# Autodesk Inventor assembly: Assembly3
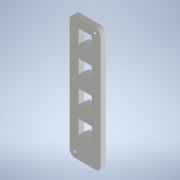
[picture p0: Inventor's stored thumbnail of the model, 180x180]
Saved by Autodesk Inventor 2020 (Build 240168000, 168)
## iProperties
Created: 2019-05-06
Part Number: Assembly3
Document SubType Name: Assembly
Designer: erwin
Author: erwin
## Documents named in this file (3)
- D:\GitHub\ProtoSwitchBoard\design\pin-header_cutter\Assembly3.iam
- D:\GitHub\ProtoSwitchBoard\design\pin-header_cutter\open_side.ipt
- D:\GitHub\ProtoSwitchBoard\design\pin-header_cutter\close_side.ipt
## Components (2 placed, 2 different names)
1. open_side:1 — Rigid:1
2. close_side:1 — Rigid:1
## Relationships (1: WeldJoint 1)
- Rigid:1 [WeldJoint]: open_side:1 ↔ close_side:1
